# Autodesk Inventor assembly: A2017_T5_12
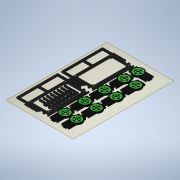
[picture p0: Inventor's stored thumbnail of the model, 180x180]
Saved by Autodesk Inventor 2022 (Build 260153000, 153)
## iProperties
Created: 2022-09-28
Part Number: A2017_T5_12
Document SubType Name: Assembly
Designer: Masato
Author: Masato
## Documents named in this file (5)
- C:\Users\ヨコオリク\Documents\CITBrains\SUSTAINA-OP\Cam\A2017_T5\A2017_T5_12.iam
- C:\Users\ヨコオリク\Documents\CITBrains\SUSTAINA-OP\Cam\DisposableBoard.ipt
- C:\Users\ヨコオリク\Documents\CITBrains\SUSTAINA-OP\UpperBody\Cockpit\Cockpit_trunk_lower_side_frame_stopper.ipt
- C:\Users\ヨコオリク\Documents\CITBrains\SUSTAINA-OP\UpperBody\Cockpit\Cockpit_circuit_board_frame.ipt
- C:\Users\ヨコオリク\Documents\CITBrains\SUSTAINA-OP\LowerBody\Leg_joint\Leg_joint_yaw_frame.ipt
## Components (20 placed, 4 different names)
1. DisposableBoard:1 — フラッシュ:1, フラッシュ:2, フラッシュ:3, フラッシュ:4, フラッシュ:5, フラッシュ:6, フラッシュ:7
2. Leg_joint_yaw_frame:9 — メイト:6, メイト:7, 正接:2
3. Cockpit_circuit_board_frame:1 — メイト:1, フラッシュ:5, フラッシュ:6, メイト:3, メイト:4, 正接:1
4. Cockpit_circuit_board_frame:2 — メイト:7
5. Cockpit_trunk_lower_side_frame_stopper:1 — メイト:2, メイト:3, メイト:4
6. Cockpit_trunk_lower_side_frame_stopper:2
7. Cockpit_trunk_lower_side_frame_stopper:3
8. Cockpit_trunk_lower_side_frame_stopper:4
9. Cockpit_trunk_lower_side_frame_stopper:5
10. Cockpit_trunk_lower_side_frame_stopper:6
11. Cockpit_trunk_lower_side_frame_stopper:7
12. Cockpit_trunk_lower_side_frame_stopper:8
13. Leg_joint_yaw_frame:1 — メイト:5, フラッシュ:7, 正接:1
14. Leg_joint_yaw_frame:2
15. Leg_joint_yaw_frame:3
16. Leg_joint_yaw_frame:4
17. Leg_joint_yaw_frame:5
18. Leg_joint_yaw_frame:6
19. Leg_joint_yaw_frame:7 — 正接:2
20. Leg_joint_yaw_frame:8
## Component patterns: (2 elements, first: Cockpit_circuit_board_frame:1), (8 elements, first: Cockpit_trunk_lower_side_frame_stopper:1), (8 elements, first: Leg_joint_yaw_frame:1)
## Relationships (16: Flush 7, Mate 7, Tangent 2)
- フラッシュ:1 [Flush]: DisposableBoard:1
- フラッシュ:2 [Flush]: DisposableBoard:1
- フラッシュ:3 [Flush]: DisposableBoard:1
- フラッシュ:4 [Flush]: DisposableBoard:1
- メイト:1 [Mate]: Cockpit_circuit_board_frame:1
- メイト:2 [Mate]: Cockpit_trunk_lower_side_frame_stopper:1
- フラッシュ:5 [Flush] (2 mm): DisposableBoard:1 ↔ Cockpit_circuit_board_frame:1
- フラッシュ:6 [Flush] (2 mm): DisposableBoard:1 ↔ Cockpit_circuit_board_frame:1
- メイト:3 [Mate] (10 mm): Cockpit_circuit_board_frame:1 ↔ Cockpit_trunk_lower_side_frame_stopper:1
- メイト:4 [Mate] (3 mm): Cockpit_circuit_board_frame:1 ↔ Cockpit_trunk_lower_side_frame_stopper:1
- メイト:5 [Mate]: Leg_joint_yaw_frame:1
- フラッシュ:7 [Flush] (2 mm): DisposableBoard:1 ↔ Leg_joint_yaw_frame:1
- 正接:1 [Tangent] (2.5 mm): Cockpit_circuit_board_frame:1 ↔ Leg_joint_yaw_frame:1
- メイト:6 [Mate]: Leg_joint_yaw_frame:9
- メイト:7 [Mate] (2.5 mm): Leg_joint_yaw_frame:9 ↔ Cockpit_circuit_board_frame:2
- 正接:2 [Tangent] (2.5 mm): Leg_joint_yaw_frame:9 ↔ Leg_joint_yaw_frame:7
